# Autodesk Inventor assembly: Assembly
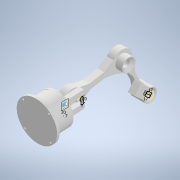
[picture p0: Inventor's stored thumbnail of the model, 180x180]
Saved by Autodesk Inventor 2022 (Build 260153000, 153)
## iProperties
Created: 2022-02-04
Part Number: Assembly
Document SubType Name: Assembly
Designer: Alexa
Author: Alexa
## Documents named in this file (6)
- C:\Users\Alexa\Documents\4TH YEAR\ROBOTICS PARTS\Assembly.iam
- C:\Users\Alexa\Documents\4TH YEAR\ROBOTICS PARTS\Base Part.ipt
- C:\Users\Alexa\Documents\4TH YEAR\ROBOTICS PARTS\BaseTop.ipt
- C:\Users\Alexa\Documents\4TH YEAR\ROBOTICS PARTS\1st-arm.ipt
- C:\Users\Alexa\Documents\4TH YEAR\ROBOTICS PARTS\2nd arm.ipt
- C:\Users\Alexa\Documents\4TH YEAR\ROBOTICS PARTS\EndConnector.ipt
## Components (5 placed, 5 different names)
1. Base Part:1 — Rotational:1
2. BaseTop:1 — Rotational:1, Rotational:2
3. 1st-arm:1 — Rotational:2, Rotational:3
4. 2nd arm:1 — Rotational:3, Rotational:4
5. EndConnector:1 — Rotational:4
## Relationships (4: RevoluteJoint 4)
- Rotational:1 [RevoluteJoint]: Base Part:1 ↔ BaseTop:1
- Rotational:2 [RevoluteJoint]: BaseTop:1 ↔ 1st-arm:1
- Rotational:3 [RevoluteJoint]: 1st-arm:1 ↔ 2nd arm:1
- Rotational:4 [RevoluteJoint]: 2nd arm:1 ↔ EndConnector:1
